# Autodesk Inventor assembly: SmartDumpster
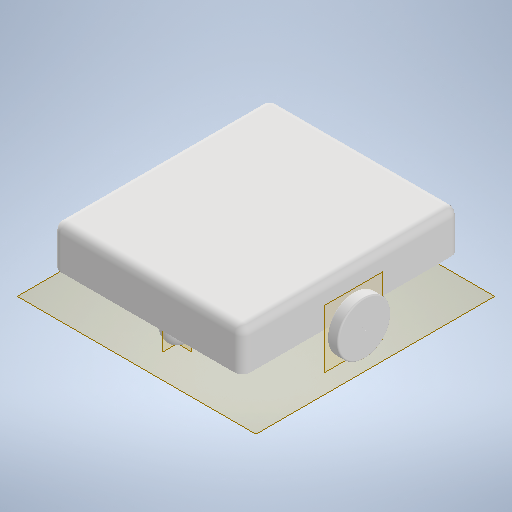
[picture p0: Inventor's stored thumbnail of the model, 512x512]
Saved by Autodesk Inventor 2025.2 (Build 292293000, 293)
## iProperties
Created: 2025-11-14
Part Number: SmartDumpster
Document SubType Name: Assembly
Designer: igles
Author: igles
## Documents named in this file (5)
- C:\Users\igles\Desktop\SmartdumpsterCAD_Simu\SmartDumpster.iam
- C:\Users\igles\Desktop\SmartdumpsterCAD_Simu\base_link.ipt
- C:\Users\igles\Desktop\SmartdumpsterCAD_Simu\caster_wheel_link.ipt
- C:\Users\igles\Desktop\SmartdumpsterCAD_Simu\wheel_left_link.ipt
- C:\Users\igles\Desktop\SmartdumpsterCAD_Simu\wheel_right_link.ipt
## Components (5 placed, 4 different names)
1. base_link:1 — Rígido:1, Rígido:2, Coincidencia:1, Coincidencia:2, Ángulo:1
2. caster_wheel_link:1 — Coincidencia:1
3. wheel_left_link:1 — Rígido:1
4. wheel_right_link:1 — Rígido:2, Tangente:1
5. caster_wheel_link:2 — Coincidencia:2
## Relationships (6: WeldJoint 2, Mate 2, Angle 1, Tangent 1)
- Rígido:1 [WeldJoint] (-40 mm): base_link:1 ↔ wheel_left_link:1
- Rígido:2 [WeldJoint] (-40 mm): base_link:1 ↔ wheel_right_link:1
- Coincidencia:1 [Mate]: base_link:1 ↔ caster_wheel_link:1
- Coincidencia:2 [Mate]: base_link:1 ↔ caster_wheel_link:2
- Ángulo:1 [Angle] (0 deg): base_link:1
- Tangente:1: wheel_right_link:1
